# Autodesk Inventor assembly: keyboard_h
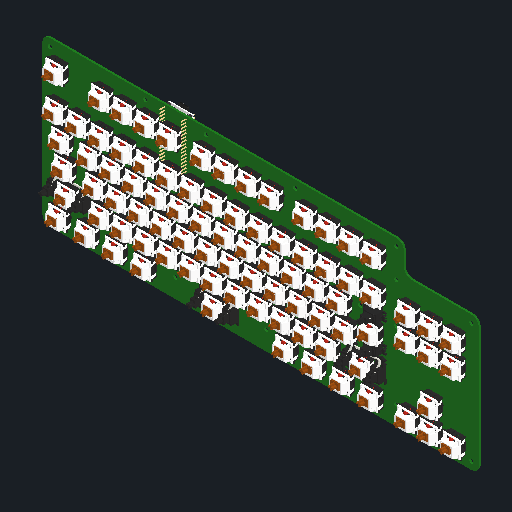
[picture p0: Inventor's stored thumbnail of the model, 512x512]
Saved by Autodesk Inventor 2022 (Build 260153000, 153)
## iProperties
Company: A Company
Created: 2021-09-12
Part Number: keyboard_h
Description: KiCad electronic assembly
Document SubType Name: Assembly
Designer: shiok
Authority: Unknown
Sending System: KiCad to STEP converter
Preprocessor: Open CASCADE STEP processor 6.9
Title: keyboard_h.step
Author: An Author
## Documents named in this file (6)
- C:\Users\shiok\Documents\GitHub\Keyboard_H\pcb\3D_model\step\keyboard_h.iam
- C:\Users\shiok\Documents\GitHub\Keyboard_H\pcb\3D_model\step\SW_Cherry_MX_PCB.iam
- C:\Users\shiok\Documents\GitHub\Keyboard_H\pcb\3D_model\step\Stabilizer_Cherry_MX_2u.iam
- C:\Users\shiok\Documents\GitHub\Keyboard_H\pcb\3D_model\step\LED_D3.0mm.iam
- C:\Users\shiok\Documents\GitHub\Keyboard_H\pcb\3D_model\step\COMPOUND_2.ipt
- C:\Users\shiok\Documents\GitHub\Keyboard_H\pcb\3D_model\step\RPiPico.iam
## Components (180 placed, 180 different names)
1. 2 [sub-assembly]
2. 3 [sub-assembly]
3. 4 [sub-assembly]
4. 5 [sub-assembly]
5. 6 [sub-assembly]
6. 7 [sub-assembly]
7. 8 [sub-assembly]
8. 9 [sub-assembly]
9. 10 [sub-assembly]
10. 11 [sub-assembly]
11. 12 [sub-assembly]
12. 13 [sub-assembly]
13. 14 [sub-assembly]
14. 15 [sub-assembly]
15. 16 [sub-assembly]
16. 17 [sub-assembly]
17. 18 [sub-assembly]
18. 19 [sub-assembly]
19. 20 [sub-assembly]
20. 21 [sub-assembly]
21. 22 [sub-assembly]
22. 23 [sub-assembly]
23. 24 [sub-assembly]
24. 25 [sub-assembly]
25. 26 [sub-assembly]
26. 27 [sub-assembly]
27. 28 [sub-assembly]
28. 29 [sub-assembly]
29. 30 [sub-assembly]
30. 31 [sub-assembly]
31. 32 [sub-assembly]
32. 33 [sub-assembly]
33. 34 [sub-assembly]
34. 35 [sub-assembly]
35. 36 [sub-assembly]
36. 37 [sub-assembly]
37. 38 [sub-assembly]
38. 39 [sub-assembly]
39. 40 [sub-assembly]
40. 41 [sub-assembly]
41. 42 [sub-assembly]
42. 43 [sub-assembly]
43. 44 [sub-assembly]
44. 45 [sub-assembly]
45. 46 [sub-assembly]
46. 47 [sub-assembly]
47. 48 [sub-assembly]
48. 49 [sub-assembly]
49. 50 [sub-assembly]
50. 51 [sub-assembly]
51. 52 [sub-assembly]
52. 53 [sub-assembly]
53. 54 [sub-assembly]
54. 55 [sub-assembly]
55. 56 [sub-assembly]
56. 57 [sub-assembly]
57. 58 [sub-assembly]
58. 59 [sub-assembly]
59. 60 [sub-assembly]
60. 61 [sub-assembly]
61. 62 [sub-assembly]
62. 63 [sub-assembly]
63. 64 [sub-assembly]
64. 65 [sub-assembly]
65. 66 [sub-assembly]
66. 67 [sub-assembly]
67. 68 [sub-assembly]
68. 69 [sub-assembly]
69. 70 [sub-assembly]
70. 71 [sub-assembly]
71. 72 [sub-assembly]
72. 73 [sub-assembly]
73. 74 [sub-assembly]
74. 75 [sub-assembly]
75. 76 [sub-assembly]
76. 77 [sub-assembly]
77. 78 [sub-assembly]
78. 79 [sub-assembly]
79. 80 [sub-assembly]
80. 81 [sub-assembly]
81. 82 [sub-assembly]
82. 83 [sub-assembly]
83. 85 [sub-assembly]
84. 86 [sub-assembly]
85. 87 [sub-assembly]
86. 88 [sub-assembly]
87. 89 [sub-assembly]
88. 90 [sub-assembly]
89. 91 [sub-assembly]
90. 92 [sub-assembly]
91. 93 [sub-assembly]
92. 95 [sub-assembly]
93. 96 [sub-assembly]
94. 97 [sub-assembly]
95. 98 [sub-assembly]
96. 99 [sub-assembly]
97. 100 [sub-assembly]
98. 101 [sub-assembly]
99. 102 [sub-assembly]
100. 103 [sub-assembly]
101. 104 [sub-assembly]
102. 105 [sub-assembly]
103. 106 [sub-assembly]
104. 107 [sub-assembly]
105. 108 [sub-assembly]
106. 109 [sub-assembly]
107. 110 [sub-assembly]
108. 111 [sub-assembly]
109. 112 [sub-assembly]
110. 113 [sub-assembly]
111. 114 [sub-assembly]
112. 115 [sub-assembly]
113. 116 [sub-assembly]
114. 117 [sub-assembly]
115. 118 [sub-assembly]
116. 119 [sub-assembly]
117. 120 [sub-assembly]
118. 121 [sub-assembly]
119. 122 [sub-assembly]
120. 123 [sub-assembly]
121. 124 [sub-assembly]
122. 125 [sub-assembly]
123. 126 [sub-assembly]
124. 127 [sub-assembly]
125. 128 [sub-assembly]
126. 129 [sub-assembly]
127. 130 [sub-assembly]
128. 131 [sub-assembly]
129. 132 [sub-assembly]
130. 133 [sub-assembly]
131. 134 [sub-assembly]
132. 135 [sub-assembly]
133. 136 [sub-assembly]
134. 137 [sub-assembly]
135. 138 [sub-assembly]
136. 139 [sub-assembly]
137. 140 [sub-assembly]
138. 141 [sub-assembly]
139. 142 [sub-assembly]
140. 143 [sub-assembly]
141. 144 [sub-assembly]
142. 145 [sub-assembly]
143. 146 [sub-assembly]
144. 147 [sub-assembly]
145. 148 [sub-assembly]
146. 149 [sub-assembly]
147. 150 [sub-assembly]
148. 151 [sub-assembly]
149. 152 [sub-assembly]
150. 153 [sub-assembly]
151. 154 [sub-assembly]
152. 155 [sub-assembly]
153. 156 [sub-assembly]
154. 157 [sub-assembly]
155. 158 [sub-assembly]
156. 159 [sub-assembly]
157. 160 [sub-assembly]
158. 161 [sub-assembly]
159. 162 [sub-assembly]
160. 163 [sub-assembly]
161. 164 [sub-assembly]
162. 165 [sub-assembly]
163. 166 [sub-assembly]
164. 167 [sub-assembly]
165. 168 [sub-assembly]
166. 169 [sub-assembly]
167. 170 [sub-assembly]
168. 171 [sub-assembly]
169. 172 [sub-assembly]
170. 173 [sub-assembly]
171. 174 [sub-assembly]
172. 175 [sub-assembly]
173. 176 [sub-assembly]
174. 177 [sub-assembly]
175. 178 [sub-assembly]
176. 179 [sub-assembly]
177. 180 [sub-assembly]
178. 181 [sub-assembly]
179. 182 — メイト:1
180. RPiPico:1 [sub-assembly] — メイト:1
## Relationships (1: Mate 1)
- メイト:1 [Mate]: 182 ↔ RPiPico:1
